# Autodesk Inventor assembly: David_v1
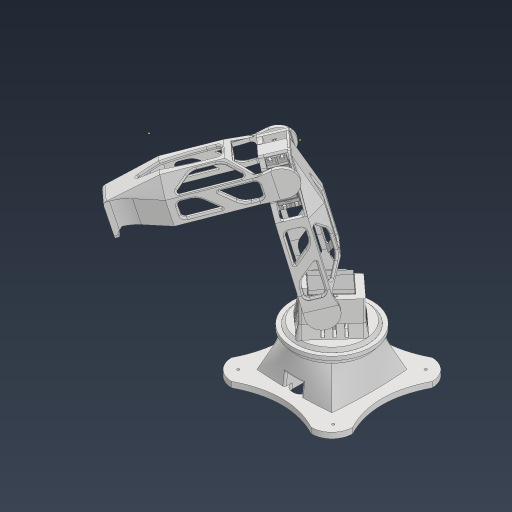
[picture p0: Inventor's stored thumbnail of the model, 512x512]
Saved by Autodesk Inventor 2024 (Build 280153000, 153)
## iProperties
Created: 2025-04-26
Part Number: David_v1
Document SubType Name: Assembly
Designer: Piter
Author: Piter
## Documents named in this file (7)
- C:\Users\Piter\OneDrive\Pulpit\Robots\david_Arm\Fresh model\Version1\David_v1.iam
- C:\Users\Piter\OneDrive\Pulpit\Robots\david_Arm\Fresh model\Version1\Fixed_mount.ipt
- C:\Users\Piter\OneDrive\Pulpit\Robots\david_Arm\Fresh model\Version1\base_support.ipt
- C:\Users\Piter\OneDrive\Pulpit\Robots\david_Arm\Fresh model\Version1\bearing_bed_arm1.ipt
- C:\Users\Piter\OneDrive\Pulpit\Robots\david_Arm\Fresh model\Version1\arm2.ipt
- C:\Users\Piter\OneDrive\Pulpit\Robots\david_Arm\Fresh model\Version1\arm_1.ipt
- C:\Users\Piter\OneDrive\Pulpit\Robots\david_Arm\Fresh model\Version1\bearing_bed_arm2_tight.ipt
## Components (6 placed, 6 different names)
1. Fixed_mount:1 — Rotational:1, Rigid:1
2. base_support:1 — Rotational:1
3. bearing_bed_arm1:1 — Rigid:1, Rotational:2
4. arm2:1 — Rotational:3
5. arm_1:1 — Rotational:2, Rigid:2
6. bearing_bed_arm2_tight:1 — Rigid:2, Rotational:3
## Relationships (5: RevoluteJoint 3, WeldJoint 2)
- Rotational:1 [RevoluteJoint]: Fixed_mount:1 ↔ base_support:1
- Rigid:1 [WeldJoint]: Fixed_mount:1 ↔ bearing_bed_arm1:1
- Rotational:2 [RevoluteJoint]: bearing_bed_arm1:1 ↔ arm_1:1
- Rigid:2 [WeldJoint]: arm_1:1 ↔ bearing_bed_arm2_tight:1
- Rotational:3 [RevoluteJoint]: arm2:1 ↔ bearing_bed_arm2_tight:1
